# Autodesk Inventor assembly: ASM Main
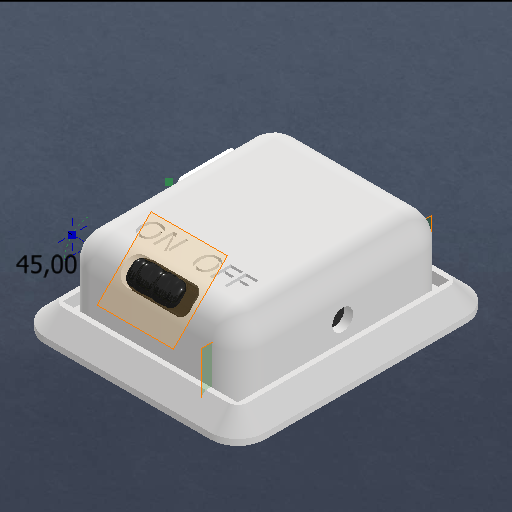
[picture p0: Inventor's stored thumbnail of the model, 512x512]
Saved by Autodesk Inventor 2025.2 (Build 292293000, 293)
## iProperties
Created: 2024-11-12
Part Number: ASM Main
Document SubType Name: Assembly
Designer: matss
Author: matss
## Documents named in this file (10)
- C:\Users\matss\Documents\.Studium\Health_Device\CAD\Wearable-Health-Device\ASM Main.iam
- C:\Users\matss\Documents\.Studium\Health_Device\CAD\Wearable-Health-Device\MCI_PCB\MCI_PCB\MCI_PCB.iam
- C:\Users\matss\Documents\.Studium\Health_Device\CAD\Wearable-Health-Device\PCB_Mount.ipt
- C:\Users\matss\Documents\.Studium\Health_Device\CAD\Wearable-Health-Device\PCB_Deckel.ipt
- C:\Users\matss\Documents\.Studium\Health_Device\CAD\Wearable-Health-Device\Schalter.ipt
- C:\Users\matss\Documents\.Studium\Health_Device\CAD\Wearable-Health-Device\Schalter_vergroeßerung.ipt
- C:\Users\matss\Documents\.Studium\Health_Device\CAD\Wearable-Health-Device\USB-C_cover.ipt
- C:\Users\matss\Documents\.Studium\Health_Device\CAD\Wearable-Health-Device\IMU_Base_T-Shirt_PCB.ipt
- C:\Users\matss\Documents\.Studium\Health_Device\CAD\Wearable-Health-Device\Batterie.ipt
- C:\Users\matss\Documents\.Studium\Health_Device\CAD\Wearable-Health-Device\Led.ipt
## Components (9 placed, 9 different names)
1. MCI_PCB:1 [sub-assembly] — Mate:4, Mate:5, Mate:6, Mate:19, Angle:1, Mate:23, Flush:11, Flush:12, Mate:24, Mate:25, Angle:2
2. PCB_Mount:1 — Mate:1, Mate:2, Mate:3, Mate:4, Mate:5, Mate:6, Mate:7, Mate:8, Flush:10, Mate:20
3. PCB_Deckel:1 — Mate:7, Mate:8, Flush:10, Mate:9, Mate:10, Mate:17, Mate:18, Mate:21, Mate:22
4. Schalter:1 — Mate:12, Mate:15, Mate:16
5. Schalter_vergroeßerung:1 — Mate:9, Mate:10, Mate:12, Mate:15, Mate:16
6. USB-C_cover:1 — Mate:17, Mate:18
7. IMU_Base_T-Shirt_PCB:1 — Mate:20, Mate:21, Mate:22
8. Batterie:1 — Mate:23, Flush:11, Flush:12
9. Led:1 — Mate:24, Mate:25, Angle:2
## Relationships (27: Mate 22, Flush 3, Angle 2)
- Mate:1: PCB_Mount:1
- Mate:2: PCB_Mount:1
- Mate:3 (20 mm): PCB_Mount:1
- Mate:4 (2.5 mm): MCI_PCB:1 ↔ PCB_Mount:1
- Mate:5: MCI_PCB:1 ↔ PCB_Mount:1
- Mate:6: MCI_PCB:1 ↔ PCB_Mount:1
- Mate:7: PCB_Mount:1 ↔ PCB_Deckel:1
- Mate:8: PCB_Mount:1 ↔ PCB_Deckel:1
- Flush:10: PCB_Mount:1 ↔ PCB_Deckel:1
- Mate:9 (0.25 mm): PCB_Deckel:1 ↔ Schalter_vergroeßerung:1
- Mate:10 (0.5 mm): PCB_Deckel:1 ↔ Schalter_vergroeßerung:1
- Mate:12: Schalter:1 ↔ Schalter_vergroeßerung:1
- Mate:15: Schalter:1 ↔ Schalter_vergroeßerung:1
- Mate:16 (0.5 mm): Schalter:1 ↔ Schalter_vergroeßerung:1
- Mate:17: PCB_Deckel:1 ↔ USB-C_cover:1
- Mate:18: PCB_Deckel:1 ↔ USB-C_cover:1
- Mate:19: MCI_PCB:1
- Angle:1 (0 deg): MCI_PCB:1
- Mate:20: PCB_Mount:1 ↔ IMU_Base_T-Shirt_PCB:1
- Mate:21 (0.25 mm): PCB_Deckel:1 ↔ IMU_Base_T-Shirt_PCB:1
- Mate:22 (0.25 mm): PCB_Deckel:1 ↔ IMU_Base_T-Shirt_PCB:1
- Mate:23 (3 mm): MCI_PCB:1 ↔ Batterie:1
- Flush:11 (8 mm): MCI_PCB:1 ↔ Batterie:1
- Flush:12: MCI_PCB:1 ↔ Batterie:1
- Mate:24: MCI_PCB:1 ↔ Led:1
- Mate:25: MCI_PCB:1 ↔ Led:1
- Angle:2 (0 deg): MCI_PCB:1 ↔ Led:1
